# Autodesk Inventor assembly: MontagemFinal
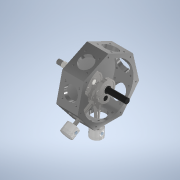
[picture p0: Inventor's stored thumbnail of the model, 180x180]
Saved by Autodesk Inventor 2021 (Build 250183000, 183)
## iProperties
Created: 2021-07-24
Part Number: MontagemFinal
Document SubType Name: Assembly
Designer: Giovanni
Author: Giovanni
## Documents named in this file (7)
- C:\Users\irineu\Documents\Inventor\MotorRadial7\MontagemFinal.iam
- C:\Users\irineu\Documents\Inventor\MotorRadial7\Peça4.ipt
- C:\Users\irineu\Documents\Inventor\Content Center Files\R2021\pt-BR\DIN BEARING(1)\DIN 625 SKF - SKF 6008.ipt
- C:\Users\irineu\Documents\Inventor\MotorRadial7\Conjunto_Virabrequim.iam
- C:\Users\irineu\Documents\Inventor\MotorRadial7\BielaMestraEquipada.iam
- C:\Users\irineu\Documents\Inventor\MotorRadial7\PistaoEquipado.iam
- C:\Users\irineu\Documents\Inventor\MotorRadial7\BielaArticuladaEquipada.iam
## Components (7 placed, 6 different names)
1. Peça4:1 — Alinhado:1, Alinhado:2, Alinhado:3, Inserir:1
2. DIN 625 SKF SKF 6008:1 — Inserir:1, Inserir:2
3. Conjunto_Virabrequim:1 [sub-assembly] — Inserir:2, Inserir:3
4. BielaMestraEquipada:1 [sub-assembly] — Inserir:3, Coincidente:1, Coincidente:2, Alinhado:4, Inserir:4
5. PistaoEquipado:1 [sub-assembly] — Coincidente:1, Coincidente:2, Alinhado:4
6. BielaArticuladaEquipada:1 [sub-assembly] — Inserir:4, Coincidente:3, Alinhado:5, Alinhado:6
7. PistaoEquipado:2 [sub-assembly] — Coincidente:3, Alinhado:5, Alinhado:6
## Relationships (13: Flush 6, Insert 4, Mate 3)
- Alinhado:1 [Flush]: Peça4:1
- Alinhado:2 [Flush]: Peça4:1
- Alinhado:3 [Flush]: Peça4:1
- Inserir:1: Peça4:1 ↔ DIN 625 SKF SKF 6008:1
- Inserir:2: DIN 625 SKF SKF 6008:1 ↔ Conjunto_Virabrequim:1
- Inserir:3: Conjunto_Virabrequim:1 ↔ BielaMestraEquipada:1
- Coincidente:1 [Mate]: BielaMestraEquipada:1 ↔ PistaoEquipado:1
- Coincidente:2 [Mate]: BielaMestraEquipada:1 ↔ PistaoEquipado:1
- Alinhado:4 [Flush]: BielaMestraEquipada:1 ↔ PistaoEquipado:1
- Inserir:4: BielaMestraEquipada:1 ↔ BielaArticuladaEquipada:1
- Coincidente:3 [Mate]: BielaArticuladaEquipada:1 ↔ PistaoEquipado:2
- Alinhado:5 [Flush]: BielaArticuladaEquipada:1 ↔ PistaoEquipado:2
- Alinhado:6 [Flush]: BielaArticuladaEquipada:1 ↔ PistaoEquipado:2
